# Autodesk Inventor assembly: Pieza_robv2
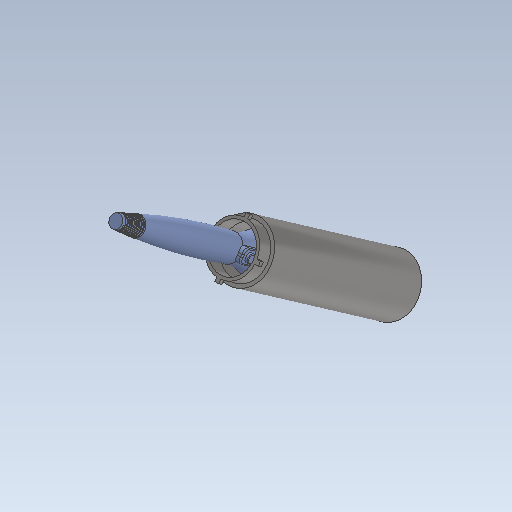
[picture p0: Inventor's stored thumbnail of the model, 512x512]
Saved by Autodesk Inventor 2026 (Build 300175000, 175)
## iProperties
Created: 2026-07-20
Part Number: Pieza_robv2
Document SubType Name: Assembly
Designer: User
Author: User
## Documents named in this file (4)
- C:\Users\User\Desktop\Pieza_robv2.iam
- C:\Users\User\Desktop\HERRAMIENTA_1.ipt
- C:\Users\User\Desktop\HERRAMIENTA_p2.ipt
- C:\Users\User\Downloads\Cautin.ipt
## Components (3 placed, 3 different names)
1. HERRAMIENTA_1:1 — Coincidencia:2
2. HERRAMIENTA_p2:1 — Coincidencia:1, Coincidencia:2
3. Cautin:1 — Coincidencia:1
## Relationships (2: Mate 2)
- Coincidencia:1 [Mate]: HERRAMIENTA_p2:1 ↔ Cautin:1
- Coincidencia:2 [Mate]: HERRAMIENTA_1:1 ↔ HERRAMIENTA_p2:1
